# Autodesk Inventor assembly: fan_assembly
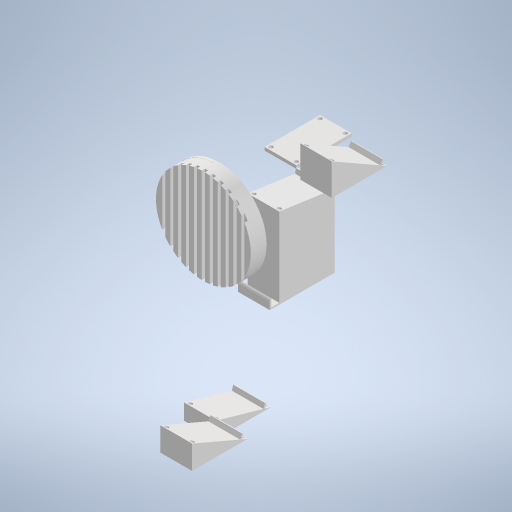
[picture p0: Inventor's stored thumbnail of the model, 512x512]
Saved by Autodesk Inventor 2023.1 (Build 271208000, 208)
## iProperties
Created: 2023-05-29
Part Number: fan_assembly
Document SubType Name: Assembly
Designer: Mansoor Lunawadi
Author: Mansoor Lunawadi
## Documents named in this file (10)
- C:\Users\67988\OneDrive\Desktop\fan_assembly.iam
- C:\Users\67988\OneDrive\Desktop\blades.ipt
- C:\Users\67988\OneDrive\Desktop\fan back.ipt
- C:\Users\67988\OneDrive\Desktop\fan front.ipt
- C:\Users\67988\OneDrive\Desktop\platform.ipt
- C:\Users\67988\OneDrive\Desktop\0_mm_slant.ipt
- C:\Users\67988\OneDrive\Desktop\5_mm_slant.ipt
- C:\Users\67988\OneDrive\Desktop\10_mm_slant.ipt
- C:\Users\67988\OneDrive\Desktop\15_mm_slant.ipt
- C:\Users\67988\OneDrive\Desktop\20_mm_slant.ipt
## Components (9 placed, 9 different names)
1. blades:1 — Mate:1, Mate:2
2. fan back:1 — Mate:2, Flush:1, Mate:3, Mate:5
3. fan front:1 — Mate:1, Flush:1, Mate:4
4. platform:1 — Mate:3, Mate:4, Mate:5, Mate:6
5. 0_mm_slant:1
6. 5_mm_slant:1 — Mate:6
7. 10_mm_slant:1
8. 15_mm_slant:1
9. 20_mm_slant:1
## Relationships (7: Mate 6, Flush 1)
- Mate:1: blades:1 ↔ fan front:1
- Mate:2: blades:1 ↔ fan back:1
- Flush:1: fan back:1 ↔ fan front:1
- Mate:3 (28 mm): fan back:1 ↔ platform:1
- Mate:4 (-57 mm): fan front:1 ↔ platform:1
- Mate:5 (-10 mm): fan back:1 ↔ platform:1
- Mate:6: platform:1 ↔ 5_mm_slant:1
